# Autodesk Inventor assembly: TR2 Arm
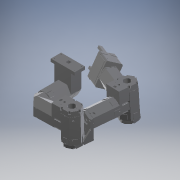
[picture p0: Inventor's stored thumbnail of the model, 180x180]
Saved by Autodesk Inventor 2017 (Build 210142000, 142)
## iProperties
Created: 2018-10-11
Part Number: TR2 Arm
Document SubType Name: Assembly
Designer: Zach
Author: Zach
## Documents named in this file (8)
- C:\Users\Dell\Documents\GitHub\tr2\Arm\Arm.iam
- C:\Users\Dell\Documents\GitHub\tr2\Arm\TARM01.ipt
- C:\Users\Dell\Documents\GitHub\tr2\Arm Actuator\Arm Actuator.iam
- C:\Users\Dell\Documents\GitHub\tr2\Arm\TARM02.ipt
- C:\Users\Dell\Documents\GitHub\tr2\Arm\TARM04.ipt
- C:\Users\Dell\Documents\GitHub\tr2\Arm\TARM08.ipt
- C:\Users\Dell\Documents\GitHub\tr2\Gripper\Gripper.iam
- C:\Users\Dell\Documents\GitHub\tr2\Arm\TARM09.ipt
## Components (13 placed, 7 different names)
1. TARM01:1 — Mate:117, Mate:118, Mate:139
2. TARM02:1 — Mate:13, Mate:106, Mate:108, Mate:109, Mate:110, Mate:140, Mate:141, Mate:142
3. TARM04:1 — Mate:113, Mate:114, Mate:145, Mate:151
4. TARM04:2 — Mate:53, Mate:112, Mate:153, Mate:157
5. TARM08:1 — Mate:108, Mate:109, Mate:110
6. Arm Actuator:1 [sub-assembly] — Mate:13, Mate:106, Mate:117, Mate:118, Mate:139
7. Arm Actuator:2 [sub-assembly] — Mate:114, Mate:143, Mate:144, Mate:145, Mate:146
8. Arm Actuator:3 [sub-assembly] — Mate:113, Mate:147, Mate:148, Mate:151, Mate:152
9. Arm Actuator:4 [sub-assembly] — Mate:153, Mate:154, Mate:155, Mate:156, Mate:157
10. Arm Actuator:5 [sub-assembly] — Mate:53, Mate:112, Mate:127, Mate:128
11. Gripper:1 [sub-assembly] — Mate:127, Mate:128
12. TARM09:1 — Mate:140, Mate:141, Mate:142, Mate:143, Mate:144, Mate:146
13. TARM09:2 — Mate:147, Mate:148, Mate:152, Mate:154, Mate:155, Mate:156
## Relationships (30: Mate 30)
- Mate:13: TARM02:1 ↔ Arm Actuator:1
- Mate:53: TARM04:2 ↔ Arm Actuator:5
- Mate:106: TARM02:1 ↔ Arm Actuator:1
- Mate:108: TARM02:1 ↔ TARM08:1
- Mate:109: TARM02:1 ↔ TARM08:1
- Mate:110: TARM02:1 ↔ TARM08:1
- Mate:112: TARM04:2 ↔ Arm Actuator:5
- Mate:113: TARM04:1 ↔ Arm Actuator:3
- Mate:114: TARM04:1 ↔ Arm Actuator:2
- Mate:117: TARM01:1 ↔ Arm Actuator:1
- Mate:118: TARM01:1 ↔ Arm Actuator:1
- Mate:127: Arm Actuator:5 ↔ Gripper:1
- Mate:128: Arm Actuator:5 ↔ Gripper:1
- Mate:139: TARM01:1 ↔ Arm Actuator:1
- Mate:140: TARM02:1 ↔ TARM09:1
- Mate:141: TARM02:1 ↔ TARM09:1
- Mate:142: TARM02:1 ↔ TARM09:1
- Mate:143: Arm Actuator:2 ↔ TARM09:1
- Mate:144: Arm Actuator:2 ↔ TARM09:1
- Mate:145: TARM04:1 ↔ Arm Actuator:2
- Mate:146: Arm Actuator:2 ↔ TARM09:1
- Mate:147: Arm Actuator:3 ↔ TARM09:2
- Mate:148: Arm Actuator:3 ↔ TARM09:2
- Mate:151: TARM04:1 ↔ Arm Actuator:3
- Mate:152: Arm Actuator:3 ↔ TARM09:2
- Mate:153: TARM04:2 ↔ Arm Actuator:4
- Mate:154: Arm Actuator:4 ↔ TARM09:2
- Mate:155: Arm Actuator:4 ↔ TARM09:2
- Mate:156: Arm Actuator:4 ↔ TARM09:2
- Mate:157: TARM04:2 ↔ Arm Actuator:4
